# Autodesk Inventor assembly: Remote Buttons Print Assembly
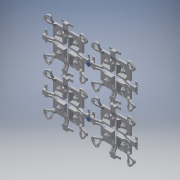
[picture p0: Inventor's stored thumbnail of the model, 180x180]
Saved by Autodesk Inventor 2016 (Build 200138000, 138)
## iProperties
Created: 2015-10-15
Part Number: Remote Buttons Print Assembly
Document SubType Name: Assembly
Designer: Sam Clay
Author: Sam Clay
## Documents named in this file (2)
- Z:\enclosure\inventor\Remote Buttons Print Assembly.iam
- Z:\enclosure\inventor\Remote Buttons.ipt
## Components (4 placed, 1 different names)
1. Remote Buttons:1
2. Remote Buttons:2
3. Remote Buttons:3
4. Remote Buttons:4
## Component patterns: (4 elements, first: Remote Buttons:1)
